# Autodesk Inventor assembly: AxisX
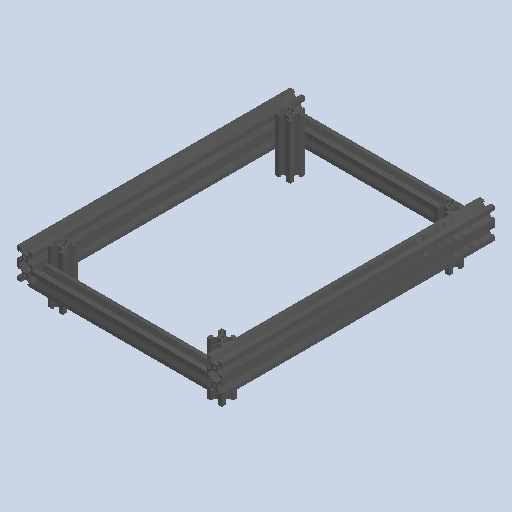
[picture p0: Inventor's stored thumbnail of the model, 512x512]
Saved by Autodesk Inventor 2024.2 (Build 282272000, 272)
## iProperties
Created: 2024-08-26
Part Number: AxisX
Document SubType Name: Assembly
Designer: Admin
Author: Admin
## Documents named in this file (4)
- C:\Users\Admin\Documents\GitHub\ManipuladorCartesiano\DiseñoMecánico\Assemblies\AxisX.iam
- C:\Users\Admin\Documents\GitHub\ManipuladorCartesiano\DiseñoMecánico\Axis\AxisX\AP-X1.ipt
- C:\Users\Admin\Documents\GitHub\ManipuladorCartesiano\DiseñoMecánico\Axis\AxisX\AP-X2.ipt
- C:\Users\Admin\Documents\GitHub\ManipuladorCartesiano\DiseñoMecánico\Axis\AxisX\AP-Support.ipt
## Components (8 placed, 3 different names)
1. AP-X1:1 — Mate:1, Flush:1, Flush:2, Mate:3, Flush:5, Flush:8, Mate:7, Flush:10, Mate:12
2. AP-X1:2 — Mate:2, Flush:3, Flush:4, Mate:4, Flush:6, Mate:6, Flush:7, Flush:9, Mate:10
3. AP-X2:1 — Mate:3, Mate:4, Flush:5, Flush:6, Mate:5, Mate:8
4. AP-X2:2 — Mate:1, Flush:1, Flush:2, Mate:2, Flush:3, Flush:4, Mate:9, Mate:11
5. AP-Support:1 — Mate:5, Mate:6, Flush:7
6. AP-Support:2 — Flush:9, Mate:9, Mate:10
7. AP-Support:3 — Flush:10, Mate:11, Mate:12
8. AP-Support:4 — Flush:8, Mate:7, Mate:8
## Relationships (22: Mate 12, Flush 10)
- Mate:1: AP-X1:1 ↔ AP-X2:2
- Flush:1: AP-X1:1 ↔ AP-X2:2
- Flush:2: AP-X1:1 ↔ AP-X2:2
- Mate:2: AP-X1:2 ↔ AP-X2:2
- Flush:3: AP-X1:2 ↔ AP-X2:2
- Flush:4: AP-X1:2 ↔ AP-X2:2
- Mate:3: AP-X1:1 ↔ AP-X2:1
- Mate:4: AP-X1:2 ↔ AP-X2:1
- Flush:5: AP-X1:1 ↔ AP-X2:1
- Flush:6: AP-X1:2 ↔ AP-X2:1
- Mate:5: AP-X2:1 ↔ AP-Support:1
- Mate:6: AP-X1:2 ↔ AP-Support:1
- Flush:7: AP-X1:2 ↔ AP-Support:1
- Flush:8: AP-X1:1 ↔ AP-Support:4
- Mate:7: AP-X1:1 ↔ AP-Support:4
- Mate:8: AP-X2:1 ↔ AP-Support:4
- Flush:9: AP-X1:2 ↔ AP-Support:2
- Mate:9: AP-X2:2 ↔ AP-Support:2
- Mate:10: AP-X1:2 ↔ AP-Support:2
- Flush:10: AP-X1:1 ↔ AP-Support:3
- Mate:11: AP-X2:2 ↔ AP-Support:3
- Mate:12: AP-X1:1 ↔ AP-Support:3
